# Autodesk Inventor assembly: Assemblage Droite
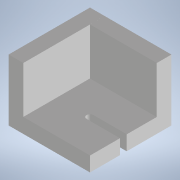
[picture p0: Inventor's stored thumbnail of the model, 180x180]
Saved by Autodesk Inventor 2020 (Build 240168000, 168)
## iProperties
Created: 2019-11-07
Part Number: Assemblage Droite
Document SubType Name: Assembly
Designer: erwan
Author: erwan
## Documents named in this file (4)
- C:\Users\erwan\Desktop\Eirbot\Coupe robotique\Table\Support de balise\Assemblage Droite.iam
- C:\Users\erwan\Desktop\Eirbot\Coupe robotique\Table\Support de balise\Support.ipt
- C:\Users\erwan\Desktop\Eirbot\Coupe robotique\Table\Support de balise\Fond.ipt
- C:\Users\erwan\Desktop\Eirbot\Coupe robotique\Table\Support de balise\Coté.ipt
## Components (3 placed, 3 different names)
1. Support:1 — Affleurement:1, Placage:1, Placage:2, Affleurement:2, Affleurement:3, Placage:3, Affleurement:4, Affleurement:5
2. Fond:1 — Placage:2, Affleurement:2, Affleurement:3
3. Coté:1 — Placage:3, Affleurement:4, Affleurement:5
## Relationships (8: Flush 5, Mate 3)
- Affleurement:1 [Flush]: Support:1
- Placage:1 [Mate]: Support:1
- Placage:2 [Mate]: Support:1 ↔ Fond:1
- Affleurement:2 [Flush]: Support:1 ↔ Fond:1
- Affleurement:3 [Flush]: Support:1 ↔ Fond:1
- Placage:3 [Mate]: Support:1 ↔ Coté:1
- Affleurement:4 [Flush]: Support:1 ↔ Coté:1
- Affleurement:5 [Flush]: Support:1 ↔ Coté:1
